# Autodesk Inventor assembly: z2cz
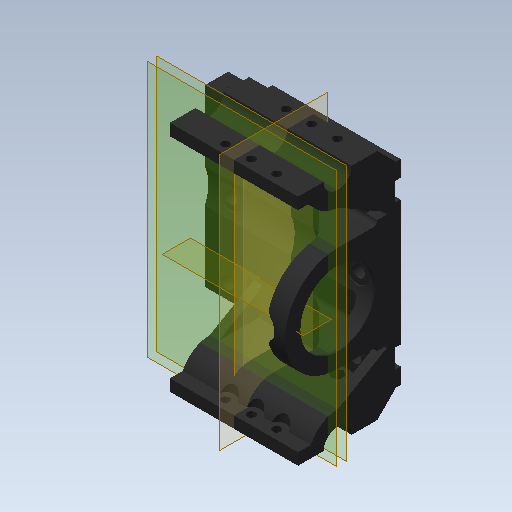
[picture p0: Inventor's stored thumbnail of the model, 512x512]
Saved by Autodesk Inventor 2020 (Build 240168000, 168)
## iProperties
Created: 2020-08-17
Part Number: z2cz
Material: Ogólny
Document SubType Name: Assembly
Designer: invin
Mass: 149.076 g
Surface Area: 435.452 cm^2
Volume: 96.74 cm^3
Density: 1.541 g/cm^3
Author: invin
## Documents named in this file (3)
- D:\KONIECTEGOKOŁCHOZU\MGR\model\Workspaces\Obszar roboczy\Całość\Cartesian2_Y\z2cz.iam
- D:\KONIECTEGOKOŁCHOZU\MGR\model\Workspaces\Obszar roboczy\OLD\Z_bearingmount.ipt
- D:\KONIECTEGOKOŁCHOZU\MGR\model\Workspaces\Obszar roboczy\OLD\ZY_rod_mount.ipt
## Components (2 placed, 2 different names)
1. Z_bearingmount:1 — Zestawiający:1, Zestawiający:2, Zestawiający:3
2. ZY_rod_mount:1 — Zestawiający:1, Zestawiający:2, Zestawiający:3
## Relationships (3: Mate 3)
- Zestawiający:1 [Mate]: Z_bearingmount:1 ↔ ZY_rod_mount:1
- Zestawiający:2 [Mate]: Z_bearingmount:1 ↔ ZY_rod_mount:1
- Zestawiający:3 [Mate]: Z_bearingmount:1 ↔ ZY_rod_mount:1
